# Autodesk Inventor assembly: 2.75 Omni AS, No Insert
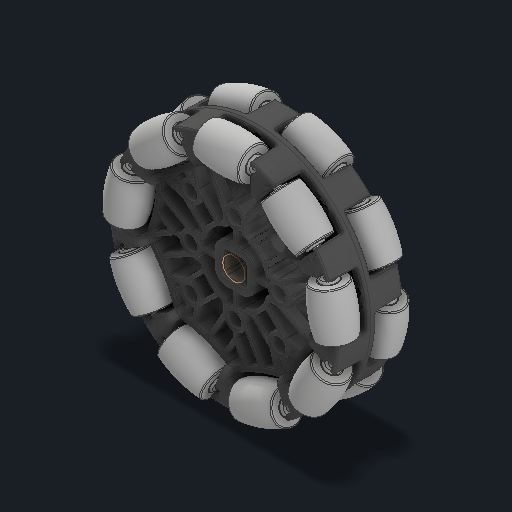
[picture p0: Inventor's stored thumbnail of the model, 512x512]
Saved by Autodesk Inventor 2025.1 (Build 291241000, 241)
## iProperties
Created: 2022-08-02
Part Number: 2.75 Omni AS, No Insert
Document SubType Name: Assembly
Designer: avere
Author: ylu12
## Documents named in this file (2)
- C:\Users\avere\VEX\High Stakes\CAD\V4\Chassis\Drivebay Right\2.75 Omni AS, No Insert.iam
- C:\Users\avere\VEX\High Stakes\CAD\V4\Chassis\Drivebay Right\2.75 Omni Antistatic.ipt
## Components (1 placed, 1 different names)
1. 2.75 Omni Antistatic:1 — Mate:8, Mate:7, Flush:4
## Relationships (3: Mate 2, Flush 1)
- Mate:8: 2.75 Omni Antistatic:1
- Mate:7: 2.75 Omni Antistatic:1
- Flush:4: 2.75 Omni Antistatic:1
